# Autodesk Inventor assembly: Assembly1
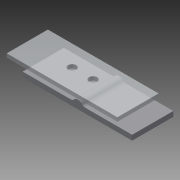
[picture p0: Inventor's stored thumbnail of the model, 180x180]
Saved by Autodesk Inventor 2013 (Build 170138000, 138)
## iProperties
Created: 2013-06-24
Part Number: Assembly1
Document SubType Name: Assembly
Designer: mvarma
Author: mvarma
## Documents named in this file (4)
- C:\Users\mvarma\Desktop\GRT 2013-2014 Gearbox\Mark 3\Test Parts\Assembly1.iam
- C:\Users\mvarma\Desktop\GRT 2013-2014 Gearbox\Mark 3\Test Parts\Test - Ball Shifting Holes.ipt
- C:\Users\mvarma\Desktop\GRT 2013-2014 Gearbox\Mark 3\Test Parts\Test - Ball Shifting Conture.ipt
- C:\Users\mvarma\Desktop\GRT 2013-2014 Gearbox\Mark 3\Ball Bearing 3- 16  in .ipt
## Components (4 placed, 3 different names)
1. Test - Ball Shifting Holes:1 — Flush:1, Flush:2, Mate:1, Mate:2
2. Test - Ball Shifting Conture:1 — Flush:1, Flush:2, Transitional:1, Transitional:2
3. Ball Bearing 3- 16  in :1 — Mate:1, Transitional:1
4. Ball Bearing 3- 16  in :2 — Mate:2, Transitional:2
## Relationships (6: Flush 2, Mate 2, Transitional 2)
- Flush:1: Test - Ball Shifting Holes:1 ↔ Test - Ball Shifting Conture:1
- Flush:2: Test - Ball Shifting Holes:1 ↔ Test - Ball Shifting Conture:1
- Mate:1: Test - Ball Shifting Holes:1 ↔ Ball Bearing 3- 16  in :1
- Mate:2: Test - Ball Shifting Holes:1 ↔ Ball Bearing 3- 16  in :2
- Transitional:1: Test - Ball Shifting Conture:1 ↔ Ball Bearing 3- 16  in :1
- Transitional:2: Test - Ball Shifting Conture:1 ↔ Ball Bearing 3- 16  in :2
